# Autodesk Inventor assembly: Rail_assy
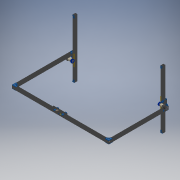
[picture p0: Inventor's stored thumbnail of the model, 180x180]
Saved by Autodesk Inventor 2019.4 (Build 234330000, 330)
## iProperties
Created: 2021-02-01
Part Number: Rail_assy
Document SubType Name: Assembly
Designer: Jorian Brusind
Author: Jorian Brusind
## Documents named in this file (7)
- C:\Users\Jorian Brusind\Documents\GitHub\PersonalProjects\HyperRail\Inventor Files\Rail_assy.iam
- C:\Users\Jorian Brusind\Documents\GitHub\PersonalProjects\HyperRail\Inventor Files\Rail_Assembly.iam
- C:\Users\Jorian Brusind\Documents\GitHub\PersonalProjects\Inventor Projects\Useful models\8020_Sets\IPT_40_Series\Extra_40_Series\HFS5-4060-4000\HFS5-4060-2125.ipt
- C:\Users\Jorian Brusind\Documents\GitHub\PersonalProjects\HyperRail\Inventor Files\YAxis_Carriage.iam
- C:\Users\Jorian Brusind\Documents\GitHub\PersonalProjects\HyperRail\Inventor Files\Small_belt_5mm_1mm.ipt
- C:\Users\Jorian Brusind\Documents\GitHub\PersonalProjects\HyperRail\Inventor Files\90deg_4040Bracket.ipt
- C:\Users\Jorian Brusind\Documents\GitHub\PersonalProjects\Inventor Projects\Useful models\8020_Sets\IPT_20_Series\Extra_20_Series\8020_14057m\14057_m.ipt
## Components (14 placed, 6 different names)
1. Rail_Assembly:1 [sub-assembly] — Mate:1, Flush:1, Flush:2, Mate:4, Mate:6, Mate:7, Flush:5, Flush:6, Mate:22, Mate:25, Flush:15, Flush:17
2. HFS5-4060-2125:1 — Mate:1, Flush:1, Flush:2, Mate:5, Flush:3, Flush:4, Mate:8, Mate:9, Mate:10, Mate:12, Mate:13, Mate:14, Flush:8, Flush:10, Mate:20, Flush:11, Mate:21, Flush:12, Mate:23, Flush:13, Flush:14, Mate:24, Mate:26, Flush:16, Mate:27, Flush:18
3. YAxis_Carriage:1 [sub-assembly] — Mate:8, Mate:9, Mate:11, Mate:15
4. Rail_Assembly:2 [sub-assembly] — Mate:5, Flush:3, Flush:4, Flush:6, Mate:16, Flush:7, Mate:17, Flush:9, Mate:18, Mate:19
5. Small_belt_5mm_1mm:1 — Mate:10, Mate:11, Mate:12
6. Small_belt_5mm_1mm:2 — Mate:13, Mate:14, Mate:15
7. 90deg_4040Bracket:1 — Mate:16, Flush:7, Flush:8
8. 90deg_4040Bracket:2 — Mate:17, Flush:9, Flush:10
9. 14057_m:1 — Mate:19, Mate:20, Flush:11
10. 14057_m:2 — Mate:18, Mate:21, Flush:12
11. 14057_m:3 — Mate:22, Mate:23, Flush:13
12. 14057_m:4 — Flush:14, Mate:24, Mate:25
13. 90deg_4040Bracket:3 — Mate:26, Flush:15, Flush:16
14. 90deg_4040Bracket:4 — Mate:27, Flush:17, Flush:18
## Relationships (43: Mate 25, Flush 18)
- Mate:1: Rail_Assembly:1 ↔ HFS5-4060-2125:1
- Flush:1: Rail_Assembly:1 ↔ HFS5-4060-2125:1
- Flush:2: Rail_Assembly:1 ↔ HFS5-4060-2125:1
- Mate:4: Rail_Assembly:1
- Mate:5: HFS5-4060-2125:1 ↔ Rail_Assembly:2
- Flush:3: HFS5-4060-2125:1 ↔ Rail_Assembly:2
- Flush:4: HFS5-4060-2125:1 ↔ Rail_Assembly:2
- Mate:6: Rail_Assembly:1
- Mate:7: Rail_Assembly:1
- Flush:5: Rail_Assembly:1
- Flush:6: Rail_Assembly:1 ↔ Rail_Assembly:2
- Mate:8 (7 mm): HFS5-4060-2125:1 ↔ YAxis_Carriage:1
- Mate:9: HFS5-4060-2125:1 ↔ YAxis_Carriage:1
- Mate:10: HFS5-4060-2125:1 ↔ Small_belt_5mm_1mm:1
- Mate:11: YAxis_Carriage:1 ↔ Small_belt_5mm_1mm:1
- Mate:12 (3.5 mm): HFS5-4060-2125:1 ↔ Small_belt_5mm_1mm:1
- Mate:13: HFS5-4060-2125:1 ↔ Small_belt_5mm_1mm:2
- Mate:14 (0.5 mm): HFS5-4060-2125:1 ↔ Small_belt_5mm_1mm:2
- Mate:15: YAxis_Carriage:1 ↔ Small_belt_5mm_1mm:2
- Mate:16: Rail_Assembly:2 ↔ 90deg_4040Bracket:1
- Flush:7: Rail_Assembly:2 ↔ 90deg_4040Bracket:1
- Flush:8: HFS5-4060-2125:1 ↔ 90deg_4040Bracket:1
- Mate:17: Rail_Assembly:2 ↔ 90deg_4040Bracket:2
- Flush:9: Rail_Assembly:2 ↔ 90deg_4040Bracket:2
- Flush:10: HFS5-4060-2125:1 ↔ 90deg_4040Bracket:2
- Mate:18: Rail_Assembly:2 ↔ 14057_m:2
- Mate:19: Rail_Assembly:2 ↔ 14057_m:1
- Mate:20: HFS5-4060-2125:1 ↔ 14057_m:1
- Flush:11: HFS5-4060-2125:1 ↔ 14057_m:1
- Mate:21: HFS5-4060-2125:1 ↔ 14057_m:2
- Flush:12: HFS5-4060-2125:1 ↔ 14057_m:2
- Mate:22: Rail_Assembly:1 ↔ 14057_m:3
- Mate:23: HFS5-4060-2125:1 ↔ 14057_m:3
- Flush:13: HFS5-4060-2125:1 ↔ 14057_m:3
- Flush:14: HFS5-4060-2125:1 ↔ 14057_m:4
- Mate:24: HFS5-4060-2125:1 ↔ 14057_m:4
- Mate:25: Rail_Assembly:1 ↔ 14057_m:4
- Mate:26: HFS5-4060-2125:1 ↔ 90deg_4040Bracket:3
- Flush:15: Rail_Assembly:1 ↔ 90deg_4040Bracket:3
- Flush:16: HFS5-4060-2125:1 ↔ 90deg_4040Bracket:3
- Mate:27: HFS5-4060-2125:1 ↔ 90deg_4040Bracket:4
- Flush:17: Rail_Assembly:1 ↔ 90deg_4040Bracket:4
- Flush:18: HFS5-4060-2125:1 ↔ 90deg_4040Bracket:4
